# Autodesk Inventor assembly: modelo_completo
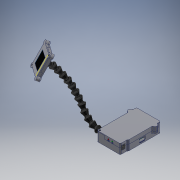
[picture p0: Inventor's stored thumbnail of the model, 180x180]
Saved by Autodesk Inventor 2019 (Build 230136000, 136)
## iProperties
Created: 2018-11-22
Part Number: modelo_completo
Material: Generic
Document SubType Name: Assembly
Designer: cadcae
Author: cadcae
## Documents named in this file (17)
- C:\Users\CADCAE\Downloads\CAD_thesis\modelo_completo.iam
- C:\Users\CADCAE\Downloads\CAD_thesis\Case2\Case_inferior_nuevo.ipt
- C:\Users\CADCAE\Downloads\CAD_thesis\PCB\tesis_schematic.iam
- C:\Users\CADCAE\Downloads\CAD_thesis\Case2\Case_superior_nuevo.ipt
- C:\Users\CADCAE\Downloads\CAD_thesis\LED\LED_3MM_ROJO.ipt
- C:\Users\CADCAE\Downloads\CAD_thesis\LED\LED_3MM_VERDE.ipt
- C:\Users\CADCAE\Downloads\CAD_thesis\Loc-line\1-4 Element.ipt
- C:\Users\CADCAE\Downloads\CAD_thesis\Inserts\94459A110_BRASS HEAT-SET INSERT FOR PLASTIC.ipt
- C:\Users\CADCAE\Downloads\CAD_thesis\Inserts\94459A120_BRASS HEAT-SET INSERT FOR PLASTIC.ipt
- C:\Users\CADCAE\Downloads\CAD_thesis\modelo_completo\Design Accelerator\Bolted Connection1.iam
- C:\Users\CADCAE\Downloads\CAD_thesis\modelo_completo\Design Accelerator\Bolted Connection2.iam
- C:\Users\CADCAE\Downloads\CAD_thesis\modelo_completo\Design Accelerator\Bolted Connection3.iam
- C:\Users\CADCAE\Downloads\CAD_thesis\Pantalla\Pantalla.ipt
- C:\Users\CADCAE\Downloads\CAD_thesis\Pantalla\Pantalla_case_superior2.ipt
- C:\Users\CADCAE\Downloads\CAD_thesis\Pantalla\pantalla_case_inferior.ipt
- C:\Users\CADCAE\Downloads\CAD_thesis\modelo_completo\Design Accelerator\Bolted Connection4.iam
- C:\Users\CADCAE\Downloads\CAD_thesis\modelo_completo\Design Accelerator\Bolted Connection5.iam
## Components (33 placed, 12 different names)
1. Case_inferior_nuevo:1 — Flush:1, Flush:2, Flush:3, Mate:1, Mate:2, Mate:3, Mate:4, Mate:5, Flush:4, Symmetry:1, Mate:11, Flush:7, Mate:13, Mate:14, Mate:17, Mate:19, Mate:21, Flush:18, Angle:5
2. tesis_schematic:1 [sub-assembly] — Mate:1, Mate:2, Mate:3, Symmetry:1
3. Case_superior_nuevo:1 — Mate:4, Mate:5, Flush:4, Mate:6, Mate:7, Angle:1, Angle:2, Mate:8, Mate:9, Mate:13, Mate:14, Flush:16, Mate:15, Flush:17, Mate:16, Angle:3, Angle:4, Mate:22
4. LED_3MM_ROJO:1 — Mate:6, Angle:2, Mate:8
5. LED_3MM_VERDE:1 — Mate:7, Angle:1, Mate:9
6. 1-4 Element:1 — Mate:10, Mate:11, Flush:7, Ball:1
7. 1-4 Element:2 — Ball:1, Ball:2
8. 1-4 Element:3 — Ball:2, Ball:3
9. 1-4 Element:4 — Ball:3, Ball:4
10. 1-4 Element:5 — Ball:4, Ball:5
11. 1-4 Element:6 — Ball:5, Ball:6
12. 1-4 Element:7 — Ball:6, Ball:7
13. 1-4 Element:8 — Ball:7, Ball:8
14. 1-4 Element:9 — Ball:8, Ball:9
15. 1-4 Element:10 — Ball:9, Ball:10
16. 94459A110_BRASS HEAT-SET INSERT FOR PLASTIC:1 — Mate:21, Flush:18, Angle:5, Mate:23
17. 94459A120_BRASS HEAT-SET INSERT FOR PLASTIC:1 — Flush:16, Mate:15, Angle:3, Mate:20
18. 94459A120_BRASS HEAT-SET INSERT FOR PLASTIC:2 — Flush:17, Mate:16, Angle:4, Mate:18
19. Bolted Connection:1 [sub-assembly] — Mate:17, Mate:18
20. Bolted Connection:2 [sub-assembly] — Mate:19, Mate:20
21. Bolted Connection:3 [sub-assembly] — Mate:22, Mate:23
22. Pantalla:1 — Mate:24, Mate:25, Mate:26
23. Pantalla_case_superior2:1 — Mate:24, Mate:25, Mate:26, Flush:22, Mate:27, Mate:28, Mate:29, Flush:25, Mate:32, Flush:26, Mate:33, Mate:34, Mate:35
24. pantalla_case_inferior:1 — Flush:22, Mate:27, Mate:28, Mate:29, Flush:23, Flush:24, Mate:36, Mate:37, Mate:38, Mate:39, Mate:40, Ball:13, Mate:41, Mate:42
25. 94459A120_BRASS HEAT-SET INSERT FOR PLASTIC:3 — Flush:24, Mate:39
26. 94459A120_BRASS HEAT-SET INSERT FOR PLASTIC:4 — Flush:25, Mate:32
27. 94459A120_BRASS HEAT-SET INSERT FOR PLASTIC:5 — Flush:26, Mate:33
28. 94459A120_BRASS HEAT-SET INSERT FOR PLASTIC:6 — Flush:23, Mate:38
29. Bolted Connection:4 [sub-assembly] — Mate:34, Mate:35, Mate:41
30. Bolted Connection:5 [sub-assembly] — Mate:36, Mate:37, Mate:42
31. 1-4 Element:11 — Ball:10, Ball:11
32. 1-4 Element:12 — Ball:11, Ball:12
33. 1-4 Element:13 — Ball:12, Mate:40, Ball:13
## Relationships (71: Mate 39, Flush 13, BallJoint 13, Angle 5, Symmetry 1)
- Flush:1: Case_inferior_nuevo:1
- Flush:2: Case_inferior_nuevo:1
- Flush:3: Case_inferior_nuevo:1
- Mate:1: Case_inferior_nuevo:1 ↔ tesis_schematic:1
- Mate:2: Case_inferior_nuevo:1 ↔ tesis_schematic:1
- Mate:3: Case_inferior_nuevo:1 ↔ tesis_schematic:1
- Mate:4: Case_inferior_nuevo:1 ↔ Case_superior_nuevo:1
- Mate:5: Case_inferior_nuevo:1 ↔ Case_superior_nuevo:1
- Flush:4: Case_inferior_nuevo:1 ↔ Case_superior_nuevo:1
- Mate:6: Case_superior_nuevo:1 ↔ LED_3MM_ROJO:1
- Mate:7: Case_superior_nuevo:1 ↔ LED_3MM_VERDE:1
- Angle:1 (0 deg): Case_superior_nuevo:1 ↔ LED_3MM_VERDE:1
- Angle:2 (0 deg): Case_superior_nuevo:1 ↔ LED_3MM_ROJO:1
- Mate:8: Case_superior_nuevo:1 ↔ LED_3MM_ROJO:1
- Mate:9: Case_superior_nuevo:1 ↔ LED_3MM_VERDE:1
- Symmetry:1: Case_inferior_nuevo:1 ↔ tesis_schematic:1
- Mate:10 (-1 mm): 1-4 Element:1
- Mate:11: Case_inferior_nuevo:1 ↔ 1-4 Element:1
- Flush:7 (2.8 mm): Case_inferior_nuevo:1 ↔ 1-4 Element:1
- Mate:13: Case_inferior_nuevo:1 ↔ Case_superior_nuevo:1
- Mate:14: Case_inferior_nuevo:1 ↔ Case_superior_nuevo:1
- Ball:1: 1-4 Element:1 ↔ 1-4 Element:2
- Ball:2: 1-4 Element:2 ↔ 1-4 Element:3
- Ball:3: 1-4 Element:3 ↔ 1-4 Element:4
- Ball:4: 1-4 Element:4 ↔ 1-4 Element:5
- Ball:5: 1-4 Element:5 ↔ 1-4 Element:6
- Ball:6: 1-4 Element:6 ↔ 1-4 Element:7
- Ball:7: 1-4 Element:7 ↔ 1-4 Element:8
- Ball:8: 1-4 Element:8 ↔ 1-4 Element:9
- Ball:9: 1-4 Element:9 ↔ 1-4 Element:10
- Flush:16: Case_superior_nuevo:1 ↔ 94459A120_BRASS HEAT-SET INSERT FOR PLASTIC:1
- Mate:15: Case_superior_nuevo:1 ↔ 94459A120_BRASS HEAT-SET INSERT FOR PLASTIC:1
- Flush:17: Case_superior_nuevo:1 ↔ 94459A120_BRASS HEAT-SET INSERT FOR PLASTIC:2
- Mate:16: Case_superior_nuevo:1 ↔ 94459A120_BRASS HEAT-SET INSERT FOR PLASTIC:2
- Angle:3 (0 deg): Case_superior_nuevo:1 ↔ 94459A120_BRASS HEAT-SET INSERT FOR PLASTIC:1
- Angle:4 (0 deg): Case_superior_nuevo:1 ↔ 94459A120_BRASS HEAT-SET INSERT FOR PLASTIC:2
- Mate:17: Case_inferior_nuevo:1 ↔ Bolted Connection:1
- Mate:18: 94459A120_BRASS HEAT-SET INSERT FOR PLASTIC:2 ↔ Bolted Connection:1
- Mate:19: Case_inferior_nuevo:1 ↔ Bolted Connection:2
- Mate:20: 94459A120_BRASS HEAT-SET INSERT FOR PLASTIC:1 ↔ Bolted Connection:2
- Mate:21: Case_inferior_nuevo:1 ↔ 94459A110_BRASS HEAT-SET INSERT FOR PLASTIC:1
- Flush:18: Case_inferior_nuevo:1 ↔ 94459A110_BRASS HEAT-SET INSERT FOR PLASTIC:1
- Angle:5 (0 deg): Case_inferior_nuevo:1 ↔ 94459A110_BRASS HEAT-SET INSERT FOR PLASTIC:1
- Mate:22: Case_superior_nuevo:1 ↔ Bolted Connection:3
- Mate:23: 94459A110_BRASS HEAT-SET INSERT FOR PLASTIC:1 ↔ Bolted Connection:3
- Mate:24: Pantalla:1 ↔ Pantalla_case_superior2:1
- Mate:25: Pantalla:1 ↔ Pantalla_case_superior2:1
- Mate:26: Pantalla:1 ↔ Pantalla_case_superior2:1
- Flush:22: Pantalla_case_superior2:1 ↔ pantalla_case_inferior:1
- Mate:27: Pantalla_case_superior2:1 ↔ pantalla_case_inferior:1
- Mate:28: Pantalla_case_superior2:1 ↔ pantalla_case_inferior:1
- Mate:29: Pantalla_case_superior2:1 ↔ pantalla_case_inferior:1
- Flush:23: pantalla_case_inferior:1 ↔ 94459A120_BRASS HEAT-SET INSERT FOR PLASTIC:6
- Flush:24: pantalla_case_inferior:1 ↔ 94459A120_BRASS HEAT-SET INSERT FOR PLASTIC:3
- Flush:25: Pantalla_case_superior2:1 ↔ 94459A120_BRASS HEAT-SET INSERT FOR PLASTIC:4
- Mate:32: Pantalla_case_superior2:1 ↔ 94459A120_BRASS HEAT-SET INSERT FOR PLASTIC:4
- Flush:26: Pantalla_case_superior2:1 ↔ 94459A120_BRASS HEAT-SET INSERT FOR PLASTIC:5
- Mate:33: Pantalla_case_superior2:1 ↔ 94459A120_BRASS HEAT-SET INSERT FOR PLASTIC:5
- Mate:34: Pantalla_case_superior2:1 ↔ Bolted Connection:4
- Mate:35: Pantalla_case_superior2:1 ↔ Bolted Connection:4
- Mate:36: pantalla_case_inferior:1 ↔ Bolted Connection:5
- Mate:37: pantalla_case_inferior:1 ↔ Bolted Connection:5
- Ball:10: 1-4 Element:10 ↔ 1-4 Element:11
- Ball:11: 1-4 Element:11 ↔ 1-4 Element:12
- Ball:12: 1-4 Element:12 ↔ 1-4 Element:13
- Mate:38: pantalla_case_inferior:1 ↔ 94459A120_BRASS HEAT-SET INSERT FOR PLASTIC:6
- Mate:39: pantalla_case_inferior:1 ↔ 94459A120_BRASS HEAT-SET INSERT FOR PLASTIC:3
- Mate:40: pantalla_case_inferior:1 ↔ 1-4 Element:13
- Ball:13: pantalla_case_inferior:1 ↔ 1-4 Element:13
- Mate:41: pantalla_case_inferior:1 ↔ Bolted Connection:4
- Mate:42: pantalla_case_inferior:1 ↔ Bolted Connection:5
